# Autodesk Inventor assembly: Baugruppe1
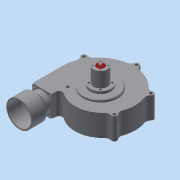
[picture p0: Inventor's stored thumbnail of the model, 180x180]
Saved by Autodesk Inventor 2018 (Build 220112000, 112)
## iProperties
Created: 2020-05-23
Part Number: Baugruppe1
Material: Generisch
Document SubType Name: Assembly
Designer: marce
Author: marce
## Documents named in this file (8)
- C:\Users\marce\OneDrive\CAD\Aluschmelzen\V2\Luefter\Baugruppe1.iam
- C:\Users\marce\OneDrive\CAD\Aluschmelzen\V2\Luefter\Lagerhalter.ipt
- C:\Users\marce\OneDrive\CAD\Aluschmelzen\V2\Luefter\Turbolader.ipt
- C:\Users\marce\OneDrive\CAD\Aluschmelzen\V2\Luefter\Gehäuse oben.ipt
- C:\Users\marce\OneDrive\CAD\Aluschmelzen\V2\Luefter\Welle.ipt
- C:\Users\marce\OneDrive\CAD\Aluschmelzen\V2\Luefter\Lager.ipt
- C:\Users\marce\OneDrive\CAD\Aluschmelzen\V2\Luefter\Gehäuse unten_1.ipt
- C:\Users\marce\OneDrive\CAD\Aluschmelzen\V2\Luefter\Rohrhalterung_2.ipt
## Components (8 placed, 7 different names)
1. Turbolader:1 — Passend:12, Passend:13
2. Lagerhalter:1 — Passend:14, Passend:15, Passend:16, Passend:17, Passend:30, Passend:31, Passend:32, Passend:33, Passend:35
3. Welle:1 — Passend:12, Passend:13, Passend:34, Passend:35
4. Lager:1 — Passend:14, Passend:15
5. Lager:2 — Passend:16, Passend:17, Passend:34
6. Gehäuse oben:2 — Fluchtend:1, Fluchtend:2, Passend:28, Passend:29, Passend:36, Passend:39
7. Gehäuse unten_1:1 — Fluchtend:1, Fluchtend:2, Passend:28, Passend:29, Passend:30, Passend:31, Passend:32, Passend:33, Passend:37, Passend:38
8. Rohrhalterung_2:1 — Passend:36, Passend:37, Passend:38, Passend:39
## Relationships (20: Mate 18, Flush 2)
- Passend:12 [Mate]: Turbolader:1 ↔ Welle:1
- Passend:13 [Mate]: Turbolader:1 ↔ Welle:1
- Passend:14 [Mate]: Lagerhalter:1 ↔ Lager:1
- Passend:15 [Mate]: Lagerhalter:1 ↔ Lager:1
- Passend:16 [Mate]: Lagerhalter:1 ↔ Lager:2
- Passend:17 [Mate]: Lagerhalter:1 ↔ Lager:2
- Fluchtend:1 [Flush]: Gehäuse oben:2 ↔ Gehäuse unten_1:1
- Fluchtend:2 [Flush]: Gehäuse oben:2 ↔ Gehäuse unten_1:1
- Passend:28 [Mate]: Gehäuse oben:2 ↔ Gehäuse unten_1:1
- Passend:29 [Mate]: Gehäuse oben:2 ↔ Gehäuse unten_1:1
- Passend:30 [Mate]: Lagerhalter:1 ↔ Gehäuse unten_1:1
- Passend:31 [Mate]: Lagerhalter:1 ↔ Gehäuse unten_1:1
- Passend:32 [Mate]: Lagerhalter:1 ↔ Gehäuse unten_1:1
- Passend:33 [Mate]: Lagerhalter:1 ↔ Gehäuse unten_1:1
- Passend:34 [Mate]: Welle:1 ↔ Lager:2
- Passend:35 [Mate]: Lagerhalter:1 ↔ Welle:1
- Passend:36 [Mate]: Gehäuse oben:2 ↔ Rohrhalterung_2:1
- Passend:37 [Mate]: Gehäuse unten_1:1 ↔ Rohrhalterung_2:1
- Passend:38 [Mate]: Gehäuse unten_1:1 ↔ Rohrhalterung_2:1
- Passend:39 [Mate]: Gehäuse oben:2 ↔ Rohrhalterung_2:1
